# Autodesk Inventor assembly: InjectorBoard
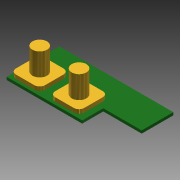
[picture p0: Inventor's stored thumbnail of the model, 180x180]
Saved by Autodesk Inventor 2014 (Build 180170000, 170)
## iProperties
Created: 2015-01-07
Part Number: InjectorBoard
Document SubType Name: Assembly
Designer: Owner
Author: Owner
## Documents named in this file (4)
- C:\Users\Owner\Documents\APC\FrontEnd\IAM\Common\InjectorBoard.iam
- C:\Users\Owner\Documents\APC\FrontEnd\IAM\Common\InjectorBoard.ipt
- C:\Users\Owner\Documents\APC\FrontEnd\IAM\Common\SMA_Up.ipt
- C:\Users\Owner\Documents\APC\FrontEnd\IAM\Common\BNC_Up.ipt
## Components (5 placed, 3 different names)
1. InjectorBoard:1 — Mate:1, Mate:2, Mate:3, Mate:4, Flush:1, Flush:2, Flush:3, Flush:4, Flush:5, Flush:6, Flush:7, Flush:8
2. SMA_Up:1 — Mate:1, Flush:6, Flush:8
3. SMA_Up:2 — Mate:2, Flush:5, Flush:7
4. BNC_Up:1 — Mate:3, Flush:1, Flush:3
5. BNC_Up:2 — Mate:4, Flush:2, Flush:4
## Relationships (12: Flush 8, Mate 4)
- Mate:1: InjectorBoard:1 ↔ SMA_Up:1
- Mate:2: InjectorBoard:1 ↔ SMA_Up:2
- Mate:3: InjectorBoard:1 ↔ BNC_Up:1
- Mate:4: InjectorBoard:1 ↔ BNC_Up:2
- Flush:1 (1.6256 mm): InjectorBoard:1 ↔ BNC_Up:1
- Flush:2 (1.6256 mm): InjectorBoard:1 ↔ BNC_Up:2
- Flush:3 (-0.762 mm): InjectorBoard:1 ↔ BNC_Up:1
- Flush:4 (24.4348 mm): InjectorBoard:1 ↔ BNC_Up:2
- Flush:5 (0.5842 mm): InjectorBoard:1 ↔ SMA_Up:2
- Flush:6 (0.5842 mm): InjectorBoard:1 ↔ SMA_Up:1
- Flush:7 (11.5062 mm): InjectorBoard:1 ↔ SMA_Up:2
- Flush:8 (-27.7622 mm): InjectorBoard:1 ↔ SMA_Up:1
